# Autodesk Inventor assembly: czlon_4_zloz_MIR1
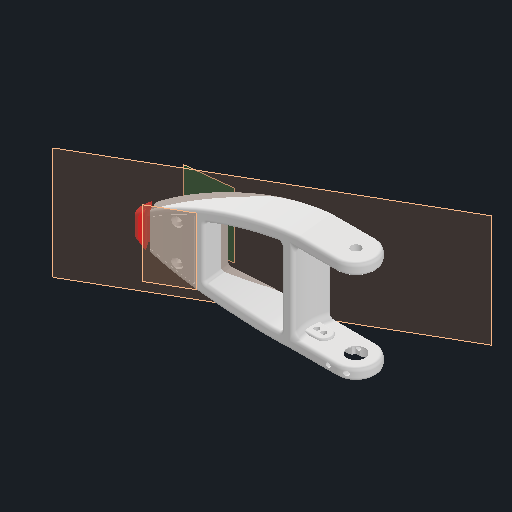
[picture p0: Inventor's stored thumbnail of the model, 512x512]
Saved by Autodesk Inventor 2023.4 (Build 274418000, 418)
## iProperties
Created: 2024-08-02
Part Number: czlon_4_zloz_MIR1
Document SubType Name: Assembly
Designer: komputer
Author: komputer
## Documents named in this file (7)
- E:\PROJECTS_REPOS\Robal-2.0\mechanics\czlon_4_zloz_MIR1.iam
- E:\PROJECTS_REPOS\Robal-2.0\mechanics\czlon4_pre_2_MIR2.ipt
- E:\PROJECTS_REPOS\Robal-2.0\mechanics\but_MIR1.ipt
- E:\PROJECTS_REPOS\Robal-2.0\mechanics\Micro Limit Switch\Micro Limit Switch_MIR1.ipt
- E:\PROJECTS_REPOS\Robal-2.0\mechanics\czlon4_pre_2_pokrywa_MIR1.ipt
- E:\PROJECTS_REPOS\Robal-2.0\mechanics\czlon4_2_wciecie_1_MIR1.ipt
- E:\PROJECTS_REPOS\Robal-2.0\mechanics\STL\podkladka_switch_MIR1.ipt
## Components (6 placed, 6 different names)
1. czlon4_pre_2_MIR2:1 — Mate:2, Mate:1, Mate:4, Mate:3, Angle:1, Mate:6, Flush:2, Angle:2, Mate:5, Mate:7, Flush:4, Mate:10, Mate:9, Mate:8, Mate:13, Mate:12, Mate:11
2. but_MIR1:1 — Mate:4, Mate:3, Angle:1
3. Micro Limit Switch_MIR1:1 — Mate:6, Flush:2, Angle:2, Mate:5, Flush:5
4. czlon4_pre_2_pokrywa_MIR1:1 — Flush:4, Mate:10, Mate:9, Mate:8, Flush:3
5. czlon4_2_wciecie_1_MIR1:1 — Mate:13, Mate:12, Mate:11
6. podkladka_switch_MIR1:1 — Flush:5
## Relationships (19: Mate 14, Flush 3, Angle 2)
- Mate:2: czlon4_pre_2_MIR2:1
- Mate:1 [Flush]: czlon4_pre_2_MIR2:1
- Mate:4 (0.2 mm): czlon4_pre_2_MIR2:1 ↔ but_MIR1:1
- Mate:3 (0.5 mm): czlon4_pre_2_MIR2:1 ↔ but_MIR1:1
- Angle:1 (0 deg): czlon4_pre_2_MIR2:1 ↔ but_MIR1:1
- Mate:6 (1.05 mm): czlon4_pre_2_MIR2:1 ↔ Micro Limit Switch_MIR1:1
- Flush:2: czlon4_pre_2_MIR2:1 ↔ Micro Limit Switch_MIR1:1
- Angle:2 (180 deg): czlon4_pre_2_MIR2:1 ↔ Micro Limit Switch_MIR1:1
- Mate:5: czlon4_pre_2_MIR2:1 ↔ Micro Limit Switch_MIR1:1
- Mate:7: czlon4_pre_2_MIR2:1
- Flush:4 (28.575 mm): czlon4_pre_2_MIR2:1 ↔ czlon4_pre_2_pokrywa_MIR1:1
- Mate:10: czlon4_pre_2_MIR2:1 ↔ czlon4_pre_2_pokrywa_MIR1:1
- Mate:9: czlon4_pre_2_MIR2:1 ↔ czlon4_pre_2_pokrywa_MIR1:1
- Mate:8: czlon4_pre_2_MIR2:1 ↔ czlon4_pre_2_pokrywa_MIR1:1
- Flush:3 [Mate] (28.75 mm): czlon4_pre_2_pokrywa_MIR1:1
- Mate:13: czlon4_pre_2_MIR2:1 ↔ czlon4_2_wciecie_1_MIR1:1
- Mate:12: czlon4_pre_2_MIR2:1 ↔ czlon4_2_wciecie_1_MIR1:1
- Mate:11: czlon4_pre_2_MIR2:1 ↔ czlon4_2_wciecie_1_MIR1:1
- Flush:5 [Mate]: Micro Limit Switch_MIR1:1 ↔ podkladka_switch_MIR1:1
